# Autodesk Inventor assembly: Модуль
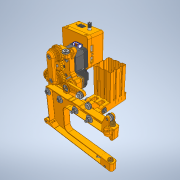
[picture p0: Inventor's stored thumbnail of the model, 180x180]
Saved by Autodesk Inventor 2021.1 (Build 251245010, 245A)
## iProperties
Created: 2026-04-18
Part Number: Модуль
Document SubType Name: Assembly
Designer: Андрей Тарасов
Author: Андрей Тарасов
## Documents named in this file (41)
- G:\04. Inventor\024. EDM 3.0\Модуль.iam
- G:\04. Inventor\024. EDM 3.0\U-подшипник.ipt
- G:\04. Inventor\024. EDM 3.0\Каркас роликов натяжителя.ipt
- G:\04. Inventor\024. EDM 3.0\Nema-17.ipt
- G:\04. Inventor\024. EDM 3.0\Ролик натяжителя.iam
- G:\04. Inventor\024. EDM 3.0\Модуль\Мастер проектирования\Цилиндрическое зубчатое зацепление1.iam
- G:\04. Inventor\024. EDM 3.0\Шестерня мотора.ipt
- G:\04. Inventor\024. EDM 3.0\Распорка роликов натяжителя.ipt
- G:\04. Inventor\024. EDM 3.0\Болт М5х35.ipt
- G:\04. Inventor\024. EDM 3.0\Гайка М5.ipt
- G:\04. Inventor\024. EDM 3.0\Рычаг натяжителя.ipt
- G:\04. Inventor\024. EDM 3.0\AS5600.ipt
- G:\04. Inventor\024. EDM 3.0\Гвоздик 3 мм.ipt
- G:\04. Inventor\024. EDM 3.0\Ограничительный стержень.ipt
- G:\04. Inventor\024. EDM 3.0\Кронштейн тянущего шаговика.ipt
- G:\04. Inventor\024. EDM 3.0\Резьбовая втулка.ipt
- G:\04. Inventor\024. EDM 3.0\Крепление модуля.ipt
- G:\04. Inventor\024. EDM 3.0\Болт М3х16.ipt
- G:\04. Inventor\024. EDM 3.0\Боковая хуйня для крепления.ipt
- G:\04. Inventor\024. EDM 3.0\Гвоздик 4х12 мм.ipt
- G:\04. Inventor\024. EDM 3.0\Шайба M5x15.ipt
- G:\04. Inventor\024. EDM 3.0\Бетонная рама.ipt
- G:\04. Inventor\024. EDM 3.0\Болт М5х30.ipt
- G:\04. Inventor\024. EDM 3.0\Подшипник 8х14х4.ipt
- G:\04. Inventor\024. EDM 3.0\Шкив рычага.ipt
- G:\04. Inventor\024. EDM 3.0\Трубка рычага.ipt
- G:\04. Inventor\024. EDM 3.0\Шпунтик магнитика.ipt
- G:\04. Inventor\024. EDM 3.0\Вал роликов натяжителя.ipt
- G:\04. Inventor\024. EDM 3.0\Проставка датчика.ipt
- G:\04. Inventor\024. EDM 3.0\Сопло фильеры.ipt
- G:\04. Inventor\024. EDM 3.0\Армирующий сопло гвоздик.ipt
- G:\04. Inventor\024. EDM 3.0\Проволока-2.ipt
- G:\04. Inventor\024. EDM 3.0\Сопло для воды.ipt
- G:\04. Inventor\024. EDM 3.0\Штырёк 4 мм.ipt
- G:\04. Inventor\024. EDM 3.0\Гайка М6.ipt
- G:\04. Inventor\024. EDM 3.0\Болт М6х40.ipt
- G:\04. Inventor\024. EDM 3.0\Шайба M6x15.ipt
- G:\04. Inventor\024. EDM 3.0\Колпачок датчика.ipt
- G:\04. Inventor\024. EDM 3.0\Корпус электроники.iam
- G:\04. Inventor\024. EDM 3.0\Ролик с шестерней (4 канала).ipt
- G:\04. Inventor\024. EDM 3.0\Уголок.ipt
## Components (93 placed, 40 different names)
1. Крепление модуля:1 — Совмещение:128, Совмещение:137, Заподлицо:41, Совмещение:215, Совмещение:216, Совмещение:217, Совмещение:218, Совмещение:221
2. Каркас роликов натяжителя:1 — Совмещение:48, Совмещение:61, Совмещение:62, Совмещение:68, Совмещение:69, Заподлицо:18, Совмещение:70, Совмещение:71, Заподлицо:19, Совмещение:72, Совмещение:73, Совмещение:88, Заподлицо:21, Совмещение:93, Совмещение:98, Совмещение:99, Совмещение:100, Заподлицо:26, Заподлицо:27, Заподлицо:28, Жесткий:24, Жесткий:25, Жесткий:26, Жесткий:27, С поворотом:2, Жесткий:33, Жесткий:34, Жесткий:35, Жесткий:36, Совмещение:149, Совмещение:150, Совмещение:151, Совмещение:167, Совмещение:180, Совмещение:181, Совмещение:184, Совмещение:185, Жесткий:60, Жесткий:61, Совмещение:190, С поворотом:70, С поворотом:71, Жесткий:68, Жесткий:69, Совмещение:194
3. Кронштейн тянущего шаговика:1 — Совмещение:93, Совмещение:96, Совмещение:106, Совмещение:107, Совмещение:109, Совмещение:110, Заподлицо:32, Совмещение:111, Совмещение:112, Заподлицо:33, Совмещение:113, Жесткий:18, Жесткий:19, Жесткий:20, Жесткий:21, Жесткий:23, Жесткий:28, Жесткий:47, Совмещение:191, Жесткий:71, Жесткий:72, Совмещение:245, Совмещение:248, Совмещение:253
4. Распорка роликов натяжителя:1 — Жесткий:64, Жесткий:65, С поворотом:72
5. Распорка роликов натяжителя:2 — Жесткий:66, Жесткий:67
6. Рычаг натяжителя:1 — Совмещение:79, Совмещение:91, Жесткий:30, Совмещение:186, Совмещение:187, С поворотом:65
7. Nema-17:1 — Совмещение:48, Совмещение:166, Совмещение:167, Заподлицо:44
8. Nema-17:2 — Совмещение:106, Совмещение:107, Совмещение:113, Совмещение:123
9. Ролик натяжителя:1 [sub-assembly] — С поворотом:71, ЗубчПер:5, С поворотом:72
10. Ролик натяжителя:2 [sub-assembly] — С поворотом:70, ЗубчПер:6
11. Ролик натяжителя:4 [sub-assembly] — Совмещение:96, Заподлицо:42, ЗубчПер:7, Заподлицо:43
12. Шестерня мотора:1 — Совмещение:61, Совмещение:62, ЗубчПер:5, ЗубчПер:6
13. Шестерня мотора:2 — Совмещение:123, Заподлицо:42, ЗубчПер:7
14. AS5600:1 — С поворотом:75, Совмещение:195, Совмещение:242, Совмещение:243
15. Цилиндрическое зубчатое зацепление:1 [sub-assembly]
16. Боковая хуйня для крепления:1 — Совмещение:128, Совмещение:129, Совмещение:137, Жесткий:48, Заподлицо:41, Совмещение:231, Совмещение:232, Совмещение:233, Совмещение:234, Совмещение:235, Совмещение:236, Совмещение:237, Совмещение:239
17. Бетонная рама:1 — Совмещение:149, Совмещение:150, Совмещение:151, Совмещение:168, Совмещение:169, Жесткий:52, Жесткий:56, Жесткий:57, Совмещение:182, Совмещение:183, Совмещение:197, Совмещение:198, С поворотом:76, Жесткий:78, Жесткий:73, Совмещение:206, Жесткий:82, Совмещение:223, Совмещение:224, Совмещение:225, Совмещение:226, Совмещение:227, Совмещение:230, Совмещение:231, Совмещение:238, Совмещение:239, Жесткий:83
18. Шкив рычага:1 — Жесткий:62, Совмещение:187
19. Трубка рычага:1 — Жесткий:63, С поворотом:4
20. Шпунтик магнитика:1 — С поворотом:4
21. Вал роликов натяжителя:1 — Жесткий:68
22. Вал роликов натяжителя:2 — Жесткий:69
23. Вал роликов натяжителя:3 — Жесткий:71, Совмещение:247
24. Вал роликов натяжителя:4 — Жесткий:72
25. Проставка датчика:1 — Совмещение:192, Совмещение:193, Совмещение:194, С поворотом:75, Совмещение:195
26. Сопло фильеры:1 — С поворотом:76
27. Сопло фильеры:2 — Совмещение:223, Совмещение:224
28. Армирующий сопло гвоздик:1 — Жесткий:73
29. Армирующий сопло гвоздик:2 — Жесткий:78
30. Проволока-2:1 — Касательность:1, Касательность:2
31. Сопло для воды:1 — Совмещение:227
32. Гайка М6:1 — Совмещение:216, Совмещение:217, Совмещение:218
33. Болт М6х40:1 — Совмещение:215, Совмещение:219, Совмещение:220
34. Шайба M6x15:1 — Совмещение:219, Совмещение:220, Совмещение:221
35. Колпачок датчика:1 — Совмещение:242, Совмещение:243
36. Корпус электроники:1 [sub-assembly] — Совмещение:245, Заподлицо:44, Совмещение:250, Совмещение:251, Совмещение:252
37. Ролик с шестерней (4 канала):1 — Совмещение:247, Заподлицо:43, Совмещение:248
38. Уголок:1 — Совмещение:250, Совмещение:251, Совмещение:252, Совмещение:253
39. Штырёк 4 мм:3 — Жесткий:82
40. Штырёк 4 мм:2 — Совмещение:206
41. Штырёк 4 мм:1 — Жесткий:83
42. Резьбовая втулка:1 — Совмещение:98, Заподлицо:28, Совмещение:144
43. Резьбовая втулка:2 — Совмещение:99, Заподлицо:27
44. Резьбовая втулка:3 — Совмещение:100, Заподлицо:26, Совмещение:125
45. Резьбовая втулка:4 — Жесткий:36, Совмещение:193
46. Резьбовая втулка:5 — Жесткий:33, Совмещение:192
47. Резьбовая втулка:6 — Жесткий:34
48. Резьбовая втулка:7 — Жесткий:35
49. Болт М3х16:1 — Жесткий:28
50. Болт М3х16:2 — Жесткий:18
51. Болт М3х16:3 — Жесткий:19, Совмещение:125
52. Болт М3х16:4 — Жесткий:23
53. Болт М3х16:5 — Жесткий:47, Совмещение:144
54. Болт М3х16:6 — Жесткий:21
55. Болт М3х16:7 — Жесткий:20
56. Болт М3х16:8 — Жесткий:25
57. Болт М3х16:9 — Жесткий:24, Совмещение:166
58. Болт М3х16:10 — Жесткий:26
59. Болт М3х16:11 — Жесткий:27
60. Болт М5х30:2 — Совмещение:232, Совмещение:233, Совмещение:234, Совмещение:238
61. Болт М5х30:3 — Совмещение:235, Совмещение:236, Совмещение:237, Совмещение:241
62. Болт М5х30:4 — Совмещение:180, Совмещение:182, Совмещение:185
63. Болт М5х30:5 — Совмещение:181, Совмещение:183, Совмещение:184
64. Болт М5х35:1 — Жесткий:64
65. Болт М5х35:2 — Жесткий:65, Совмещение:190
66. Болт М5х35:3 — Жесткий:66
67. Болт М5х35:4 — Жесткий:67, Совмещение:191
68. Гайка М5:1 — Совмещение:68, Совмещение:69, Заподлицо:18
69. Гайка М5:2 — Совмещение:70, Совмещение:71, Заподлицо:19
70. Гайка М5:3 — Совмещение:109, Совмещение:110, Заподлицо:32
71. Гайка М5:4 — Совмещение:111, Совмещение:112, Заподлицо:33
72. Гайка М5:5 — Жесткий:54, Совмещение:241
73. Гайка М5:6 — Жесткий:55
74. Гайка М5:8 — Жесткий:58
75. Гайка М5:9 — Жесткий:59
76. Гвоздик 3 мм:1 — С поворотом:2
77. Гвоздик 3 мм:2 — Жесткий:30
78. Гвоздик 4х12 мм:1 — Жесткий:41
79. Гвоздик 4х12 мм:2 — Жесткий:42
80. Шайба M5x15:1 — Жесткий:52, Жесткий:55
81. Шайба M5x15:2 — Жесткий:54, Совмещение:230
82. Шайба M5x15:4 — Жесткий:56, Жесткий:58
83. Шайба M5x15:5 — Жесткий:57, Жесткий:59
84. Ограничительный стержень:1 — Совмещение:88, Заподлицо:21
85. U-подшипник:9 — Совмещение:225, Совмещение:226
86. Подшипник 8х14х4:1 — Жесткий:60, Жесткий:63
87. Подшипник 8х14х4:2 — Жесткий:61, С поворотом:65
88. Подшипник 8х14х4:3 — Совмещение:186, Жесткий:62
89. U-подшипник:8 — Совмещение:197, Совмещение:198, Касательность:1
90. U-подшипник:3 — Совмещение:168, Совмещение:169, Касательность:2
91. U-подшипник:4 — Совмещение:72, Совмещение:73
92. U-подшипник:6 — Совмещение:79, Совмещение:91, Жесткий:41
93. U-подшипник:7 — Совмещение:129, Жесткий:42, Жесткий:48
## Relationships (153: Mate 86, WeldJoint 42, Flush 12, RevoluteJoint 8, RelateRotation 3, Tangent 2)
- Совмещение:48 [Mate]: Каркас роликов натяжителя:1 ↔ Nema-17:1
- Совмещение:61 [Mate]: Каркас роликов натяжителя:1 ↔ Шестерня мотора:1
- Совмещение:62 [Mate] (1 mm): Каркас роликов натяжителя:1 ↔ Шестерня мотора:1
- Совмещение:68 [Mate]: Каркас роликов натяжителя:1 ↔ Гайка М5:1
- Совмещение:69 [Mate]: Каркас роликов натяжителя:1 ↔ Гайка М5:1
- Заподлицо:18 [Flush]: Каркас роликов натяжителя:1 ↔ Гайка М5:1
- Совмещение:70 [Mate]: Каркас роликов натяжителя:1 ↔ Гайка М5:2
- Совмещение:71 [Mate]: Каркас роликов натяжителя:1 ↔ Гайка М5:2
- Заподлицо:19 [Flush]: Каркас роликов натяжителя:1 ↔ Гайка М5:2
- Совмещение:72 [Mate]: Каркас роликов натяжителя:1 ↔ U-подшипник:4
- Совмещение:73 [Mate]: Каркас роликов натяжителя:1 ↔ U-подшипник:4
- Совмещение:79 [Mate] (1 mm): Рычаг натяжителя:1 ↔ U-подшипник:6
- Совмещение:88 [Mate]: Каркас роликов натяжителя:1 ↔ Ограничительный стержень:1
- Заподлицо:21 [Flush]: Каркас роликов натяжителя:1 ↔ Ограничительный стержень:1
- Совмещение:91 [Mate]: Рычаг натяжителя:1 ↔ U-подшипник:6
- Совмещение:93 [Mate]: Каркас роликов натяжителя:1 ↔ Кронштейн тянущего шаговика:1
- Совмещение:96 [Mate]: Кронштейн тянущего шаговика:1 ↔ Ролик натяжителя:4
- Совмещение:98 [Mate]: Каркас роликов натяжителя:1 ↔ Резьбовая втулка:1
- Совмещение:99 [Mate]: Каркас роликов натяжителя:1 ↔ Резьбовая втулка:2
- Совмещение:100 [Mate]: Каркас роликов натяжителя:1 ↔ Резьбовая втулка:3
- Заподлицо:26 [Flush]: Каркас роликов натяжителя:1 ↔ Резьбовая втулка:3
- Заподлицо:27 [Flush]: Каркас роликов натяжителя:1 ↔ Резьбовая втулка:2
- Заподлицо:28 [Flush]: Каркас роликов натяжителя:1 ↔ Резьбовая втулка:1
- Совмещение:106 [Mate]: Кронштейн тянущего шаговика:1 ↔ Nema-17:2
- Совмещение:107 [Mate]: Кронштейн тянущего шаговика:1 ↔ Nema-17:2
- Совмещение:109 [Mate]: Кронштейн тянущего шаговика:1 ↔ Гайка М5:3
- Совмещение:110 [Mate]: Кронштейн тянущего шаговика:1 ↔ Гайка М5:3
- Заподлицо:32 [Flush]: Кронштейн тянущего шаговика:1 ↔ Гайка М5:3
- Совмещение:111 [Mate]: Кронштейн тянущего шаговика:1 ↔ Гайка М5:4
- Совмещение:112 [Mate]: Кронштейн тянущего шаговика:1 ↔ Гайка М5:4
- Заподлицо:33 [Flush]: Кронштейн тянущего шаговика:1 ↔ Гайка М5:4
- Совмещение:113 [Mate]: Кронштейн тянущего шаговика:1 ↔ Nema-17:2
- Совмещение:123 [Mate]: Nema-17:2 ↔ Шестерня мотора:2
- Жесткий:18 [WeldJoint]: Кронштейн тянущего шаговика:1 ↔ Болт М3х16:2
- Жесткий:19 [WeldJoint]: Кронштейн тянущего шаговика:1 ↔ Болт М3х16:3
- Жесткий:20 [WeldJoint]: Кронштейн тянущего шаговика:1 ↔ Болт М3х16:7
- Жесткий:21 [WeldJoint]: Кронштейн тянущего шаговика:1 ↔ Болт М3х16:6
- Жесткий:23 [WeldJoint]: Кронштейн тянущего шаговика:1 ↔ Болт М3х16:4
- Жесткий:24 [WeldJoint]: Каркас роликов натяжителя:1 ↔ Болт М3х16:9
- Жесткий:25 [WeldJoint]: Каркас роликов натяжителя:1 ↔ Болт М3х16:8
- Жесткий:26 [WeldJoint]: Каркас роликов натяжителя:1 ↔ Болт М3х16:10
- Жесткий:27 [WeldJoint]: Каркас роликов натяжителя:1 ↔ Болт М3х16:11
- Жесткий:28 [WeldJoint]: Кронштейн тянущего шаговика:1 ↔ Болт М3х16:1
- Совмещение:125 [Mate]: Резьбовая втулка:3 ↔ Болт М3х16:3
- Совмещение:128 [Mate] (0.05 mm): Крепление модуля:1 ↔ Боковая хуйня для крепления:1
- Совмещение:129 [Mate]: Боковая хуйня для крепления:1 ↔ U-подшипник:7
- Жесткий:30 [WeldJoint]: Рычаг натяжителя:1 ↔ Гвоздик 3 мм:2
- С поворотом:2 [RevoluteJoint] (2 mm): Каркас роликов натяжителя:1 ↔ Гвоздик 3 мм:1
- Жесткий:33 [WeldJoint]: Каркас роликов натяжителя:1 ↔ Резьбовая втулка:5
- Жесткий:34 [WeldJoint]: Каркас роликов натяжителя:1 ↔ Резьбовая втулка:6
- Жесткий:35 [WeldJoint]: Каркас роликов натяжителя:1 ↔ Резьбовая втулка:7
- Жесткий:36 [WeldJoint]: Каркас роликов натяжителя:1 ↔ Резьбовая втулка:4
- Совмещение:137 [Mate]: Крепление модуля:1 ↔ Боковая хуйня для крепления:1
- Жесткий:41 [WeldJoint]: Гвоздик 4х12 мм:1 ↔ U-подшипник:6
- Жесткий:42 [WeldJoint]: Гвоздик 4х12 мм:2 ↔ U-подшипник:7
- Жесткий:47 [WeldJoint]: Кронштейн тянущего шаговика:1 ↔ Болт М3х16:5
- Совмещение:144 [Mate]: Резьбовая втулка:1 ↔ Болт М3х16:5
- Совмещение:149 [Mate]: Каркас роликов натяжителя:1 ↔ Бетонная рама:1
- Совмещение:150 [Mate]: Каркас роликов натяжителя:1 ↔ Бетонная рама:1
- Совмещение:151 [Mate]: Каркас роликов натяжителя:1 ↔ Бетонная рама:1
- Жесткий:48 [WeldJoint]: Боковая хуйня для крепления:1 ↔ U-подшипник:7
- Совмещение:166 [Mate]: Nema-17:1 ↔ Болт М3х16:9
- Совмещение:167 [Mate]: Каркас роликов натяжителя:1 ↔ Nema-17:1
- Заподлицо:41 [Flush] (1 mm): Крепление модуля:1 ↔ Боковая хуйня для крепления:1
- Совмещение:168 [Mate]: Бетонная рама:1 ↔ U-подшипник:3
- Совмещение:169 [Mate]: Бетонная рама:1 ↔ U-подшипник:3
- Жесткий:52 [WeldJoint]: Бетонная рама:1 ↔ Шайба M5x15:1
- Жесткий:54 [WeldJoint]: Гайка М5:5 ↔ Шайба M5x15:2
- Жесткий:55 [WeldJoint]: Гайка М5:6 ↔ Шайба M5x15:1
- Жесткий:56 [WeldJoint]: Бетонная рама:1 ↔ Шайба M5x15:4
- Жесткий:57 [WeldJoint]: Бетонная рама:1 ↔ Шайба M5x15:5
- Жесткий:58 [WeldJoint]: Гайка М5:8 ↔ Шайба M5x15:4
- Жесткий:59 [WeldJoint]: Гайка М5:9 ↔ Шайба M5x15:5
- Совмещение:180 [Mate]: Каркас роликов натяжителя:1 ↔ Болт М5х30:4
- Совмещение:181 [Mate]: Каркас роликов натяжителя:1 ↔ Болт М5х30:5
- Совмещение:182 [Mate]: Бетонная рама:1 ↔ Болт М5х30:4
- Совмещение:183 [Mate]: Бетонная рама:1 ↔ Болт М5х30:5
- Совмещение:184 [Mate]: Каркас роликов натяжителя:1 ↔ Болт М5х30:5
- Совмещение:185 [Mate]: Каркас роликов натяжителя:1 ↔ Болт М5х30:4
- Жесткий:60 [WeldJoint]: Каркас роликов натяжителя:1 ↔ Подшипник 8х14х4:1
- Жесткий:61 [WeldJoint]: Каркас роликов натяжителя:1 ↔ Подшипник 8х14х4:2
- Совмещение:186 [Mate]: Рычаг натяжителя:1 ↔ Подшипник 8х14х4:3
- Жесткий:62 [WeldJoint]: Шкив рычага:1 ↔ Подшипник 8х14х4:3
- Совмещение:187 [Mate] (0.5 mm): Рычаг натяжителя:1 ↔ Шкив рычага:1
- Жесткий:63 [WeldJoint] (3 mm): Трубка рычага:1 ↔ Подшипник 8х14х4:1
- С поворотом:4 [RevoluteJoint]: Трубка рычага:1 ↔ Шпунтик магнитика:1
- С поворотом:65 [RevoluteJoint] (1 mm): Рычаг натяжителя:1 ↔ Подшипник 8х14х4:2
- Заподлицо:42 [Flush]: Ролик натяжителя:4 ↔ Шестерня мотора:2
- Жесткий:64 [WeldJoint]: Распорка роликов натяжителя:1 ↔ Болт М5х35:1
- Жесткий:65 [WeldJoint]: Распорка роликов натяжителя:1 ↔ Болт М5х35:2
- Совмещение:190 [Mate]: Каркас роликов натяжителя:1 ↔ Болт М5х35:2
- Жесткий:66 [WeldJoint]: Распорка роликов натяжителя:2 ↔ Болт М5х35:3
- Жесткий:67 [WeldJoint]: Распорка роликов натяжителя:2 ↔ Болт М5х35:4
- Совмещение:191 [Mate]: Кронштейн тянущего шаговика:1 ↔ Болт М5х35:4
- С поворотом:70 [RevoluteJoint]: Каркас роликов натяжителя:1 ↔ Ролик натяжителя:2
- С поворотом:71 [RevoluteJoint]: Каркас роликов натяжителя:1 ↔ Ролик натяжителя:1
- ЗубчПер:5 [RelateRotation] (1.4 ul): Ролик натяжителя:1 ↔ Шестерня мотора:1
- ЗубчПер:6 [RelateRotation] (1.4 ul): Ролик натяжителя:2 ↔ Шестерня мотора:1
- С поворотом:72 [RevoluteJoint]: Распорка роликов натяжителя:1 ↔ Ролик натяжителя:1
- Жесткий:68 [WeldJoint]: Каркас роликов натяжителя:1 ↔ Вал роликов натяжителя:1
- Жесткий:69 [WeldJoint]: Каркас роликов натяжителя:1 ↔ Вал роликов натяжителя:2
- Жесткий:71 [WeldJoint]: Кронштейн тянущего шаговика:1 ↔ Вал роликов натяжителя:3
- Жесткий:72 [WeldJoint]: Кронштейн тянущего шаговика:1 ↔ Вал роликов натяжителя:4
- ЗубчПер:7 [RelateRotation] (1.4 ul): Ролик натяжителя:4 ↔ Шестерня мотора:2
- Совмещение:192 [Mate]: Проставка датчика:1 ↔ Резьбовая втулка:5
- Совмещение:193 [Mate]: Проставка датчика:1 ↔ Резьбовая втулка:4
- Совмещение:194 [Mate]: Каркас роликов натяжителя:1 ↔ Проставка датчика:1
- С поворотом:75 [RevoluteJoint]: AS5600:1 ↔ Проставка датчика:1
- Совмещение:195 [Mate]: AS5600:1 ↔ Проставка датчика:1
- Совмещение:197 [Mate]: Бетонная рама:1 ↔ U-подшипник:8
- Совмещение:198 [Mate] (0.5 mm): Бетонная рама:1 ↔ U-подшипник:8
- С поворотом:76 [RevoluteJoint]: Бетонная рама:1 ↔ Сопло фильеры:1
- Жесткий:78 [WeldJoint]: Бетонная рама:1 ↔ Армирующий сопло гвоздик:2
- Жесткий:73 [WeldJoint]: Бетонная рама:1 ↔ Армирующий сопло гвоздик:1
- Касательность:1 [Tangent] (-1 mm): Проволока-2:1 ↔ U-подшипник:8
- Касательность:2 [Tangent] (-1 mm): Проволока-2:1 ↔ U-подшипник:3
- Совмещение:206 [Mate]: Бетонная рама:1 ↔ Штырёк 4 мм:2
- Жесткий:82 [WeldJoint]: Бетонная рама:1 ↔ Штырёк 4 мм:3
- Совмещение:215 [Mate]: Крепление модуля:1 ↔ Болт М6х40:1
- Совмещение:216 [Mate]: Крепление модуля:1 ↔ Гайка М6:1
- Совмещение:217 [Mate]: Крепление модуля:1 ↔ Гайка М6:1
- Совмещение:218 [Mate]: Крепление модуля:1 ↔ Гайка М6:1
- Совмещение:219 [Mate]: Болт М6х40:1 ↔ Шайба M6x15:1
- Совмещение:220 [Mate]: Болт М6х40:1 ↔ Шайба M6x15:1
- Совмещение:221 [Mate]: Крепление модуля:1 ↔ Шайба M6x15:1
- Совмещение:223 [Mate]: Бетонная рама:1 ↔ Сопло фильеры:2
- Совмещение:224 [Mate]: Бетонная рама:1 ↔ Сопло фильеры:2
- Совмещение:225 [Mate]: Бетонная рама:1 ↔ U-подшипник:9
- Совмещение:226 [Mate] (0.5 mm): Бетонная рама:1 ↔ U-подшипник:9
- Совмещение:227 [Mate]: Бетонная рама:1 ↔ Сопло для воды:1
- Совмещение:230 [Mate]: Бетонная рама:1 ↔ Шайба M5x15:2
- Совмещение:231 [Mate]: Боковая хуйня для крепления:1 ↔ Бетонная рама:1
- Совмещение:232 [Mate]: Боковая хуйня для крепления:1 ↔ Болт М5х30:2
- Совмещение:233 [Mate]: Боковая хуйня для крепления:1 ↔ Болт М5х30:2
- Совмещение:234 [Mate]: Боковая хуйня для крепления:1 ↔ Болт М5х30:2
- Совмещение:235 [Mate]: Боковая хуйня для крепления:1 ↔ Болт М5х30:3
- Совмещение:236 [Mate]: Боковая хуйня для крепления:1 ↔ Болт М5х30:3
- Совмещение:237 [Mate]: Боковая хуйня для крепления:1 ↔ Болт М5х30:3
- Совмещение:238 [Mate]: Бетонная рама:1 ↔ Болт М5х30:2
- Совмещение:239 [Mate]: Боковая хуйня для крепления:1 ↔ Бетонная рама:1
- Совмещение:241 [Mate]: Болт М5х30:3 ↔ Гайка М5:5
- Жесткий:83 [WeldJoint]: Бетонная рама:1 ↔ Штырёк 4 мм:1
- Совмещение:242 [Mate]: AS5600:1 ↔ Колпачок датчика:1
- Совмещение:243 [Mate]: AS5600:1 ↔ Колпачок датчика:1
- Совмещение:245 [Mate] (0.3 mm): Кронштейн тянущего шаговика:1 ↔ Корпус электроники:1
- Совмещение:247 [Mate]: Вал роликов натяжителя:3 ↔ Ролик с шестерней (4 канала):1
- Заподлицо:43 [Flush]: Ролик натяжителя:4 ↔ Ролик с шестерней (4 канала):1
- Совмещение:248 [Mate]: Кронштейн тянущего шаговика:1 ↔ Ролик с шестерней (4 канала):1
- Заподлицо:44 [Flush]: Nema-17:1 ↔ Корпус электроники:1
- Совмещение:250 [Mate]: Корпус электроники:1 ↔ Уголок:1
- Совмещение:251 [Mate]: Корпус электроники:1 ↔ Уголок:1
- Совмещение:252 [Mate]: Корпус электроники:1 ↔ Уголок:1
- Совмещение:253 [Mate]: Кронштейн тянущего шаговика:1 ↔ Уголок:1
